# Autodesk Inventor assembly: FInished_Assembly_Mk
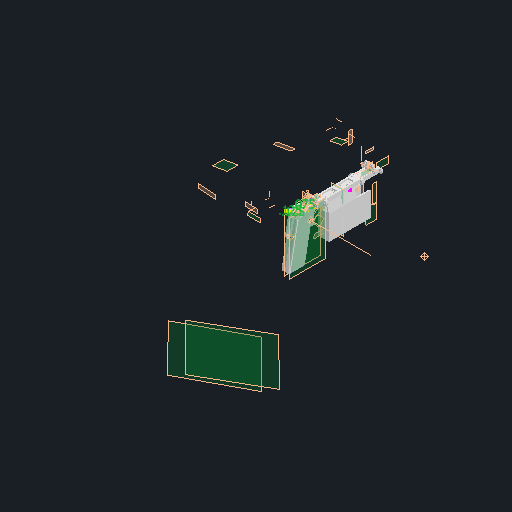
[picture p0: Inventor's stored thumbnail of the model, 512x512]
Saved by Autodesk Inventor 2024.1 (Build 281209000, 209)
## iProperties
Created: 2023-08-18
Part Number: FInished_Assembly_Mk
Document SubType Name: Assembly
Designer: Eleanor
Author: Eleanor
## Documents named in this file (8)
- C:\Users\Eleanor\Documents\Inventor\4.5mm ERS\FInished_Assembly_Mk.iam
- C:\Users\Eleanor\Documents\Inventor\4.5mm ERS\DoubleLengthCarrier.iam
- C:\Users\Eleanor\Documents\Inventor\4.5mm ERS\SlottedCarrierFull.ipt
- C:\Users\Eleanor\Documents\Inventor\4.5mm ERS\CapacitorBank.ipt.iam
- C:\Users\Eleanor\Documents\Inventor\4.5mm ERS\WireBarrelComponent.iam
- C:\Users\Eleanor\Documents\Inventor\4.5mm ERS\TestAssembly_02.iam
- GripAssembly MK.001.iam
- CapacitorBank.ipt
## Components (5 placed, 5 different names)
1. DoubleLengthCarrier:1 [sub-assembly] — Mate:7, Mate:8, Mate:12, Mate:27, Mate:28, Mate:29, Mate:30, Mate:31
2. SlottedCarrierFull:1 — Mate:5, Mate:6, Mate:7, Mate:8, Mate:9, Mate:11, Mate:12, Mate:13, Mate:14, Mate:15
3. CapacitorBank.ipt:1 [sub-assembly] — Mate:27, Mate:28
4. WireBarrelComponent:1 [sub-assembly] — Mate:5, Mate:6, Mate:11, Mate:13, Mate:14, Mate:15
5. GripAssembly MK.001:1 [sub-assembly] — Mate:29, Mate:30, Mate:31
## Relationships (15: Mate 15)
- Mate:5: SlottedCarrierFull:1 ↔ WireBarrelComponent:1
- Mate:6: SlottedCarrierFull:1 ↔ WireBarrelComponent:1
- Mate:7: DoubleLengthCarrier:1 ↔ SlottedCarrierFull:1
- Mate:8: DoubleLengthCarrier:1 ↔ SlottedCarrierFull:1
- Mate:9: SlottedCarrierFull:1
- Mate:11: SlottedCarrierFull:1 ↔ WireBarrelComponent:1
- Mate:12: DoubleLengthCarrier:1 ↔ SlottedCarrierFull:1
- Mate:13: SlottedCarrierFull:1 ↔ WireBarrelComponent:1
- Mate:14: SlottedCarrierFull:1 ↔ WireBarrelComponent:1
- Mate:15: SlottedCarrierFull:1 ↔ WireBarrelComponent:1
- Mate:27: DoubleLengthCarrier:1 ↔ CapacitorBank.ipt:1
- Mate:28: DoubleLengthCarrier:1 ↔ CapacitorBank.ipt:1
- Mate:29: DoubleLengthCarrier:1 ↔ GripAssembly MK.001:1
- Mate:30: DoubleLengthCarrier:1 ↔ GripAssembly MK.001:1
- Mate:31: DoubleLengthCarrier:1 ↔ GripAssembly MK.001:1
